# Autodesk Inventor assembly: Montagem1
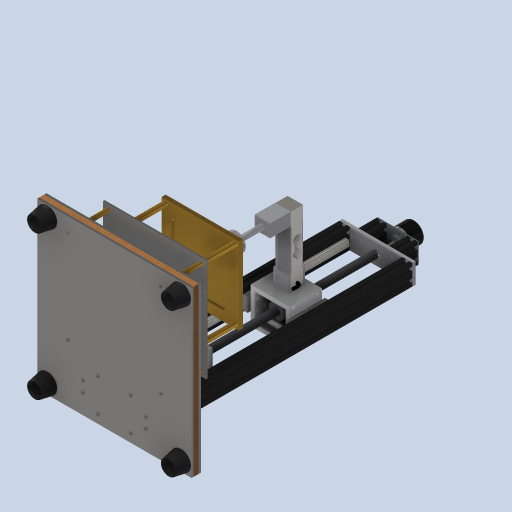
[picture p0: Inventor's stored thumbnail of the model, 512x512]
Saved by Autodesk Inventor 2023 (Build 270158000, 158)
## iProperties
Created: 2023-03-18
Part Number: Montagem1
Document SubType Name: Assembly
Designer: Mateus
Mass: 15449.6 g
Surface Area: 13309.4 cm^2
Volume: 3131.3 cm^3
Author: Mateus
## Documents named in this file (40)
- C:\Users\mateus\OneDrive - Fundação Salvador Arena\#TCC Texturômetro\1- Desenho mecânico\1-Modelagem\Texturômetro.iam
- C:\Users\mateus\OneDrive - Fundação Salvador Arena\#TCC Texturômetro\1- Desenho mecânico\1-Modelagem\Base.ipt
- C:\Users\mateus\OneDrive - Fundação Salvador Arena\#TCC Texturômetro\1- Desenho mecânico\1-Modelagem\Eixo roscado.ipt
- C:\Users\mateus\OneDrive - Fundação Salvador Arena\#TCC Texturômetro\1- Desenho mecânico\1-Modelagem\Motor.ipt
- C:\Users\mateus\OneDrive - Fundação Salvador Arena\#TCC Texturômetro\1- Desenho mecânico\1-Modelagem\Suporte do motor.ipt
- C:\Users\mateus\OneDrive - Fundação Salvador Arena\#TCC Texturômetro\1- Desenho mecânico\1-Modelagem\Sustentação motor.ipt
- C:\Users\mateus\OneDrive - Fundação Salvador Arena\#TCC Texturômetro\1- Desenho mecânico\1-Modelagem\Espaçador do motor.ipt
- C:\Users\mateus\OneDrive - Fundação Salvador Arena\#TCC Texturômetro\1- Desenho mecânico\1-Modelagem\Suporte inferior do eixo.ipt
- C:\Users\mateus\OneDrive - Fundação Salvador Arena\#TCC Texturômetro\1- Desenho mecânico\1-Modelagem\Suporte superior do eixo.ipt
- C:\Users\mateus\OneDrive - Fundação Salvador Arena\#TCC Texturômetro\1- Desenho mecânico\1-Modelagem\Suporte da base de apoio.ipt
- C:\Users\mateus\OneDrive - Fundação Salvador Arena\#TCC Texturômetro\1- Desenho mecânico\1-Modelagem\Base de apoio.ipt
- C:\Users\mateus\OneDrive - Fundação Salvador Arena\#TCC Texturômetro\1- Desenho mecânico\1-Modelagem\Guia do eixo roscado.ipt
- C:\Users\mateus\OneDrive - Fundação Salvador Arena\#TCC Texturômetro\1- Desenho mecânico\1-Modelagem\Suporte guia.ipt
- C:\Users\mateus\OneDrive - Fundação Salvador Arena\#TCC Texturômetro\1- Desenho mecânico\1-Modelagem\Guia do trilho.ipt
- C:\Users\mateus\OneDrive - Fundação Salvador Arena\#TCC Texturômetro\1- Desenho mecânico\1-Modelagem\Frente da caixa de sustentação.ipt
- C:\Users\mateus\OneDrive - Fundação Salvador Arena\#TCC Texturômetro\1- Desenho mecânico\1-Modelagem\Traseira da caixa de sustentação.ipt
- C:\Users\mateus\OneDrive - Fundação Salvador Arena\#TCC Texturômetro\1- Desenho mecânico\1-Modelagem\Suporte da célula de carga.ipt
- C:\Users\mateus\OneDrive - Fundação Salvador Arena\#TCC Texturômetro\1- Desenho mecânico\1-Modelagem\Suporte da probe.ipt
- C:\Users\mateus\OneDrive - Fundação Salvador Arena\#TCC Texturômetro\1- Desenho mecânico\1-Modelagem\Trilho.ipt
- C:\Users\mateus\OneDrive - Fundação Salvador Arena\#TCC Texturômetro\1- Desenho mecânico\1-Modelagem\Suporte base da mesa.ipt
- C:\Users\mateus\OneDrive - Fundação Salvador Arena\#TCC Texturômetro\1- Desenho mecânico\1-Modelagem\Suporte da mesa.ipt
- C:\Users\mateus\OneDrive - Fundação Salvador Arena\#TCC Texturômetro\1- Desenho mecânico\1-Modelagem\Placa da mesa.ipt
- C:\Users\mateus\OneDrive - Fundação Salvador Arena\#TCC Texturômetro\1- Desenho mecânico\1-Modelagem\Suporte mesa.ipt
- C:\Users\mateus\OneDrive - Fundação Salvador Arena\#TCC Texturômetro\1- Desenho mecânico\1-Modelagem\Probe.ipt
- C:\Users\mateus\OneDrive - Fundação Salvador Arena\#TCC Texturômetro\1- Desenho mecânico\1-Modelagem\Base madeira.ipt
- C:\Users\mateus\OneDrive - Fundação Salvador Arena\#TCC Texturômetro\1- Desenho mecânico\1-Modelagem\Perfil aluminio.ipt
- C:\Users\mateus\OneDrive - Fundação Salvador Arena\#TCC Texturômetro\1- Desenho mecânico\1-Modelagem\Lateral da caixa de sustentação.ipt
- C:\Users\mateus\OneDrive - Fundação Salvador Arena\#TCC Texturômetro\1- Desenho mecânico\1-Modelagem\Pés.ipt
- C:\Users\mateus\OneDrive - Fundação Salvador Arena\#TCC Texturômetro\1- Desenho mecânico\1-Modelagem\Perfil aluminio 2.ipt
- C:\Users\mateus\OneDrive - Fundação Salvador Arena\#TCC Texturômetro\1- Desenho mecânico\1-Modelagem\Suporte Encoder.ipt
- C:\Users\mateus\OneDrive - Fundação Salvador Arena\#TCC Texturômetro\1- Desenho mecânico\1-Modelagem\Encoder.ipt
- C:\Users\mateus\OneDrive - Fundação Salvador Arena\#TCC Texturômetro\1- Desenho mecânico\1-Modelagem\GLX-150_1.ipt
- C:\Users\mateus\OneDrive - Fundação Salvador Arena\#TCC Texturômetro\1- Desenho mecânico\1-Modelagem\Texturômetro\AIP\FEA\eaa23tyn4.fins
- C:\Users\mateus\OneDrive - Fundação Salvador Arena\#TCC Texturômetro\1- Desenho mecânico\1-Modelagem\Texturômetro\AIP\FEA\eaa23tyo0.fsat
- C:\Users\mateus\OneDrive - Fundação Salvador Arena\#TCC Texturômetro\1- Desenho mecânico\1-Modelagem\Texturômetro\AIP\FEA\eaa23tyo0.ftes
- C:\Users\mateus\OneDrive - Fundação Salvador Arena\#TCC Texturômetro\1- Desenho mecânico\1-Modelagem\Texturômetro\AIP\FEA\eaa23tyo0.fwiz
- C:\Users\mateus\OneDrive - Fundação Salvador Arena\#TCC Texturômetro\1- Desenho mecânico\1-Modelagem\Texturômetro\AIP\FEA\eaa23tytc.fmsh
- C:\Users\mateus\OneDrive - Fundação Salvador Arena\#TCC Texturômetro\1- Desenho mecânico\1-Modelagem\Texturômetro\AIP\FEA\ehg7firvk.fres
- C:\Users\mateus\OneDrive - Fundação Salvador Arena\#TCC Texturômetro\1- Desenho mecânico\1-Modelagem\Texturômetro\AIP\FEA\ei38k6pxc.fmsh
- C:\Users\mateus\OneDrive - Fundação Salvador Arena\#TCC Texturômetro\1- Desenho mecânico\1-Modelagem\Texturômetro\AIP\FEA\ei38k6pxd.fres
## Components (55 placed, 31 different names)
1. Base:1 — Coincidente:13, Coincidente:17, Alinhado:12, Coincidente:27, Coincidente:28, Coincidente:29, Coincidente:30, Coincidente:48, Alinhado:28, Alinhado:29, Coincidente:269, Alinhado:84, Coincidente:273, Alinhado:86, Coincidente:275, Flush:104, Mate:298
2. Eixo roscado:1 — Coincidente:13, Coincidente:49, Coincidente:248, Mate:285, Mate:293, Mate:294, Mate:296
3. Motor:1 — Mate:291, Mate:292, Angle:1, Mate:293, Mate:296
4. Suporte do motor:1 — Coincidente:31, Coincidente:32, Coincidente:33, Coincidente:34, Coincidente:35, Coincidente:36, Coincidente:37, Coincidente:38, Coincidente:39, Alinhado:22, Mate:117, Mate:291, Mate:292, Angle:1, Angle:2
5. Sustentação motor:1 — Coincidente:29, Coincidente:34, Mate:117
6. Sustentação motor:2 — Coincidente:27, Coincidente:33
7. Sustentação motor:3 — Coincidente:30, Coincidente:32
8. Sustentação motor:4 — Coincidente:28, Coincidente:31
9. Espaçador do motor:1 — Coincidente:35, Alinhado:19, Alinhado:20, Coincidente:39, Coincidente:41
10. Espaçador do motor:2 — Coincidente:36, Alinhado:20, Alinhado:21
11. Espaçador do motor:3 — Coincidente:38, Alinhado:19
12. Espaçador do motor:4 — Coincidente:37, Alinhado:21
13. Suporte inferior do eixo:1 — Alinhado:22, Coincidente:41, Mate:294
14. Suporte superior do eixo:1 — Coincidente:248, Alinhado:91, Coincidente:278, Mate:307, Mate:308, Mate:309, Mate:310, Mate:311, Mate:312
15. Suporte da base de apoio:1 — Coincidente:45, Alinhado:25, Alinhado:26
16. Suporte da base de apoio:2 — Alinhado:25, Coincidente:47, Coincidente:48, Mate:119
17. Suporte da base de apoio:3 — Coincidente:44, Alinhado:27
18. Suporte da base de apoio:4 — Coincidente:43, Alinhado:26, Alinhado:27
19. Base de apoio:1 — Coincidente:43, Coincidente:44, Coincidente:45, Coincidente:47, Alinhado:28, Alinhado:29, Alinhado:61, Alinhado:62, Mate:119, Mate:121
20. Guia do eixo roscado:1 — Coincidente:49, Coincidente:50, Coincidente:51
21. Suporte guia:1 — Coincidente:50, Coincidente:51, Mate:284, Flush:100
22. Guia do trilho:1 — Mate:60, Coincidente:206, Alinhado:74
23. Guia do trilho:2 — Mate:60, Flush:30, Coincidente:205, Alinhado:74, Alinhado:75, Coincidente:208, Mate:279
24. Guia do trilho:3 — Mate:61, Alinhado:72, Alinhado:73
25. Guia do trilho:4 — Mate:61, Flush:30, Alinhado:72, Alinhado:73, Coincidente:204, Alinhado:75, Mate:280, Flush:99
26. Frente da caixa de sustentação:2 — Mate:115, Coincidente:126, Flush:96, Flush:97, Mate:283, Angle:3
27. Traseira da caixa de sustentação:2 — Flush:94, Flush:95, Mate:281, Mate:282, Mate:284, Flush:100
28. Suporte da célula de carga:1 — Mate:115, Coincidente:126, Angle:3, Mate:319, Flush:105, Mate:320
29. Suporte da probe:1 — Mate:295, Mate:297, Mate:321, Flush:106, Mate:322
30. Trilho:1 — Alinhado:58, Alinhado:59, Coincidente:205, Coincidente:206, Coincidente:208, Coincidente:269, Coincidente:276
31. Trilho:2 — Alinhado:58, Alinhado:59, Coincidente:204, Coincidente:277, Alinhado:90
32. Suporte base da mesa:1 — Coincidente:106, Coincidente:107, Coincidente:108, Coincidente:109, Coincidente:110, Alinhado:61, Alinhado:62, Coincidente:111, Coincidente:112, Coincidente:113
33. Suporte da mesa:1 — Coincidente:108, Flush:67, Flush:68, Mate:125
34. Suporte da mesa:2 — Coincidente:106, Coincidente:110, Flush:68, Mate:123, Mate:124
35. Suporte da mesa:3 — Coincidente:109, Flush:66, Flush:67
36. Suporte da mesa:4 — Coincidente:107, Flush:66, Mate:122
37. Placa da mesa:1 — Coincidente:111, Coincidente:112, Coincidente:113
38. Suporte mesa:1 — Flush:69, Flush:70, Mate:121, Mate:122, Mate:123, Mate:124
39. Suporte mesa:2 — Flush:69, Flush:70, Mate:125
40. Probe:1 — Mate:295, Mate:297
41. Base madeira:1 — Alinhado:84, Alinhado:85, Coincidente:272, Coincidente:273, Alinhado:86, Alinhado:87, Flush:98, Angle:2, Mate:303, Mate:305
42. Base:2 — Alinhado:85, Coincidente:272, Alinhado:87, Mate:286, Mate:288, Mate:289, Mate:299, Mate:300, Mate:301, Mate:302, Mate:304
43. Perfil aluminio:1 — Alinhado:88, Alinhado:89, Coincidente:276, Flush:98, Mate:285
44. Perfil aluminio:2 — Alinhado:88, Alinhado:89, Coincidente:275, Coincidente:277, Alinhado:90, Alinhado:91, Coincidente:278
45. Lateral da caixa de sustentação:1 — Mate:279, Flush:92, Flush:93, Flush:94, Flush:95, Mate:281, Flush:96, Flush:97, Mate:283
46. Lateral da caixa de sustentação:2 — Mate:280, Flush:92, Flush:93, Mate:282, Flush:99
47. Pés:1 — Mate:300, Mate:305
48. Pés:2 — Mate:288, Flush:101, Mate:301, Mate:303
49. Pés:3 — Mate:286, Mate:298, Mate:299, Mate:306
50. Pés:4 — Mate:289, Flush:101, Flush:104, Mate:290, Mate:302, Mate:304
51. Perfil aluminio 2:1 — Mate:307, Mate:310, Mate:311, Mate:313, Mate:314
52. Perfil aluminio 2:2 — Mate:308, Mate:309, Mate:312, Mate:315
53. Suporte Encoder:1 — Mate:313, Mate:314, Mate:315, Mate:316, Mate:317, Mate:318
54. Encoder:1 — Mate:316, Mate:317, Mate:318
55. GLX-150_1:1 — Mate:319, Flush:105, Mate:320, Mate:321, Flush:106, Mate:322
## Relationships (146: Mate 98, Flush 45, Angle 3)
- Coincidente:13 [Mate] (-150 mm): Base:1 ↔ Eixo roscado:1
- Coincidente:17 [Mate]: Base:1
- Alinhado:12 [Flush]: Base:1
- Coincidente:27 [Mate]: Base:1 ↔ Sustentação motor:2
- Coincidente:28 [Mate]: Base:1 ↔ Sustentação motor:4
- Coincidente:29 [Mate]: Base:1 ↔ Sustentação motor:1
- Coincidente:30 [Mate]: Base:1 ↔ Sustentação motor:3
- Coincidente:31 [Mate]: Suporte do motor:1 ↔ Sustentação motor:4
- Coincidente:32 [Mate]: Suporte do motor:1 ↔ Sustentação motor:3
- Coincidente:33 [Mate]: Suporte do motor:1 ↔ Sustentação motor:2
- Coincidente:34 [Mate]: Suporte do motor:1 ↔ Sustentação motor:1
- Coincidente:35 [Mate]: Suporte do motor:1 ↔ Espaçador do motor:1
- Coincidente:36 [Mate]: Suporte do motor:1 ↔ Espaçador do motor:2
- Coincidente:37 [Mate]: Suporte do motor:1 ↔ Espaçador do motor:4
- Coincidente:38 [Mate]: Suporte do motor:1 ↔ Espaçador do motor:3
- Alinhado:19 [Flush]: Espaçador do motor:1 ↔ Espaçador do motor:3
- Alinhado:20 [Flush]: Espaçador do motor:1 ↔ Espaçador do motor:2
- Alinhado:21 [Flush]: Espaçador do motor:2 ↔ Espaçador do motor:4
- Coincidente:39 [Mate]: Suporte do motor:1 ↔ Espaçador do motor:1
- Alinhado:22 [Flush]: Suporte do motor:1 ↔ Suporte inferior do eixo:1
- Coincidente:41 [Mate]: Espaçador do motor:1 ↔ Suporte inferior do eixo:1
- Coincidente:43 [Mate]: Suporte da base de apoio:4 ↔ Base de apoio:1
- Coincidente:44 [Mate]: Suporte da base de apoio:3 ↔ Base de apoio:1
- Coincidente:45 [Mate]: Suporte da base de apoio:1 ↔ Base de apoio:1
- Alinhado:25 [Flush]: Suporte da base de apoio:1 ↔ Suporte da base de apoio:2
- Alinhado:26 [Flush]: Suporte da base de apoio:1 ↔ Suporte da base de apoio:4
- Alinhado:27 [Flush]: Suporte da base de apoio:3 ↔ Suporte da base de apoio:4
- Coincidente:47 [Mate]: Suporte da base de apoio:2 ↔ Base de apoio:1
- Coincidente:48 [Mate]: Base:1 ↔ Suporte da base de apoio:2
- Alinhado:28 [Flush] (50 mm): Base:1 ↔ Base de apoio:1
- Alinhado:29 [Flush] (18.1 mm): Base:1 ↔ Base de apoio:1
- Coincidente:49 [Mate]: Eixo roscado:1 ↔ Guia do eixo roscado:1
- Coincidente:50 [Mate]: Guia do eixo roscado:1 ↔ Suporte guia:1
- Coincidente:51 [Mate]: Guia do eixo roscado:1 ↔ Suporte guia:1
- Mate:60 (3 mm): Guia do trilho:1 ↔ Guia do trilho:2
- Mate:61 (3 mm): Guia do trilho:3 ↔ Guia do trilho:4
- Flush:30: Guia do trilho:2 ↔ Guia do trilho:4
- Alinhado:58 [Flush]: Trilho:1 ↔ Trilho:2
- Alinhado:59 [Flush]: Trilho:1 ↔ Trilho:2
- Coincidente:106 [Mate]: Suporte base da mesa:1 ↔ Suporte da mesa:2
- Coincidente:107 [Mate]: Suporte base da mesa:1 ↔ Suporte da mesa:4
- Coincidente:108 [Mate]: Suporte base da mesa:1 ↔ Suporte da mesa:1
- Coincidente:109 [Mate]: Suporte base da mesa:1 ↔ Suporte da mesa:3
- Coincidente:110 [Mate]: Suporte base da mesa:1 ↔ Suporte da mesa:2
- Alinhado:61 [Flush] (25 mm): Base de apoio:1 ↔ Suporte base da mesa:1
- Alinhado:62 [Flush] (25 mm): Base de apoio:1 ↔ Suporte base da mesa:1
- Coincidente:111 [Mate]: Suporte base da mesa:1 ↔ Placa da mesa:1
- Coincidente:112 [Mate]: Suporte base da mesa:1 ↔ Placa da mesa:1
- Coincidente:113 [Mate]: Suporte base da mesa:1 ↔ Placa da mesa:1
- Mate:115: Frente da caixa de sustentação:2 ↔ Suporte da célula de carga:1
- Mate:117: Suporte do motor:1 ↔ Sustentação motor:1
- Mate:119: Suporte da base de apoio:2 ↔ Base de apoio:1
- Flush:66: Suporte da mesa:3 ↔ Suporte da mesa:4
- Flush:67: Suporte da mesa:1 ↔ Suporte da mesa:3
- Flush:68: Suporte da mesa:1 ↔ Suporte da mesa:2
- Flush:69: Suporte mesa:1 ↔ Suporte mesa:2
- Flush:70: Suporte mesa:1 ↔ Suporte mesa:2
- Mate:121: Base de apoio:1 ↔ Suporte mesa:1
- Mate:122: Suporte da mesa:4 ↔ Suporte mesa:1
- Mate:123: Suporte da mesa:2 ↔ Suporte mesa:1
- Mate:124: Suporte da mesa:2 ↔ Suporte mesa:1
- Mate:125: Suporte da mesa:1 ↔ Suporte mesa:2
- Coincidente:126 [Mate]: Frente da caixa de sustentação:2 ↔ Suporte da célula de carga:1
- Alinhado:72 [Flush]: Guia do trilho:3 ↔ Guia do trilho:4
- Alinhado:73 [Flush]: Guia do trilho:3 ↔ Guia do trilho:4
- Coincidente:204 [Mate]: Guia do trilho:4 ↔ Trilho:2
- Coincidente:205 [Mate]: Guia do trilho:2 ↔ Trilho:1
- Coincidente:206 [Mate]: Guia do trilho:1 ↔ Trilho:1
- Alinhado:74 [Flush]: Guia do trilho:1 ↔ Guia do trilho:2
- Alinhado:75 [Flush]: Guia do trilho:2 ↔ Guia do trilho:4
- Coincidente:208 [Mate]: Guia do trilho:2 ↔ Trilho:1
- Coincidente:248 [Mate]: Eixo roscado:1 ↔ Suporte superior do eixo:1
- Coincidente:269 [Mate] (12.5 mm): Base:1 ↔ Trilho:1
- Alinhado:84 [Flush]: Base:1 ↔ Base madeira:1
- Alinhado:85 [Flush]: Base madeira:1 ↔ Base:2
- Coincidente:272 [Mate]: Base madeira:1 ↔ Base:2
- Coincidente:273 [Mate]: Base:1 ↔ Base madeira:1
- Alinhado:86 [Flush]: Base:1 ↔ Base madeira:1
- Alinhado:87 [Flush]: Base madeira:1 ↔ Base:2
- Alinhado:88 [Flush]: Perfil aluminio:1 ↔ Perfil aluminio:2
- Alinhado:89 [Flush]: Perfil aluminio:1 ↔ Perfil aluminio:2
- Coincidente:275 [Mate]: Base:1 ↔ Perfil aluminio:2
- Coincidente:276 [Mate]: Trilho:1 ↔ Perfil aluminio:1
- Coincidente:277 [Mate]: Trilho:2 ↔ Perfil aluminio:2
- Alinhado:90 [Flush] (14 mm): Trilho:2 ↔ Perfil aluminio:2
- Alinhado:91 [Flush]: Suporte superior do eixo:1 ↔ Perfil aluminio:2
- Coincidente:278 [Mate]: Suporte superior do eixo:1 ↔ Perfil aluminio:2
- Mate:279: Guia do trilho:2 ↔ Lateral da caixa de sustentação:1
- Mate:280: Guia do trilho:4 ↔ Lateral da caixa de sustentação:2
- Flush:92: Lateral da caixa de sustentação:1 ↔ Lateral da caixa de sustentação:2
- Flush:93: Lateral da caixa de sustentação:1 ↔ Lateral da caixa de sustentação:2
- Flush:94: Traseira da caixa de sustentação:2 ↔ Lateral da caixa de sustentação:1
- Flush:95: Traseira da caixa de sustentação:2 ↔ Lateral da caixa de sustentação:1
- Mate:281: Traseira da caixa de sustentação:2 ↔ Lateral da caixa de sustentação:1
- Mate:282: Traseira da caixa de sustentação:2 ↔ Lateral da caixa de sustentação:2
- Flush:96: Frente da caixa de sustentação:2 ↔ Lateral da caixa de sustentação:1
- Flush:97: Frente da caixa de sustentação:2 ↔ Lateral da caixa de sustentação:1
- Mate:283: Frente da caixa de sustentação:2 ↔ Lateral da caixa de sustentação:1
- Mate:284: Suporte guia:1 ↔ Traseira da caixa de sustentação:2
- Flush:98 (28.4 mm): Base madeira:1 ↔ Perfil aluminio:1
- Flush:99 (5.25 mm): Guia do trilho:4 ↔ Lateral da caixa de sustentação:2
- Mate:285 (51 mm): Eixo roscado:1 ↔ Perfil aluminio:1
- Flush:100 (9.25 mm): Suporte guia:1 ↔ Traseira da caixa de sustentação:2
- Mate:286: Base:2 ↔ Pés:3
- Mate:288: Base:2 ↔ Pés:2
- Mate:289: Base:2 ↔ Pés:4
- Flush:101: Pés:2 ↔ Pés:4
- Flush:104: Base:1 ↔ Pés:4
- Mate:290: Pés:4
- Mate:291: Motor:1 ↔ Suporte do motor:1
- Mate:292: Motor:1 ↔ Suporte do motor:1
- Angle:1 (0 deg): Motor:1 ↔ Suporte do motor:1
- Mate:293: Eixo roscado:1 ↔ Motor:1
- Mate:294: Eixo roscado:1 ↔ Suporte inferior do eixo:1
- Angle:2 (0 deg): Suporte do motor:1 ↔ Base madeira:1
- Mate:295: Suporte da probe:1 ↔ Probe:1
- Mate:296 (8 mm): Eixo roscado:1 ↔ Motor:1
- Angle:3 (0 deg): Frente da caixa de sustentação:2 ↔ Suporte da célula de carga:1
- Mate:297: Suporte da probe:1 ↔ Probe:1
- Mate:298: Base:1 ↔ Pés:3
- Mate:299: Base:2 ↔ Pés:3
- Mate:300: Base:2 ↔ Pés:1
- Mate:301: Base:2 ↔ Pés:2
- Mate:302: Base:2 ↔ Pés:4
- Mate:303: Base madeira:1 ↔ Pés:2
- Mate:304: Base:2 ↔ Pés:4
- Mate:305: Base madeira:1 ↔ Pés:1
- Mate:306: Pés:3
- Mate:307: Suporte superior do eixo:1 ↔ Perfil aluminio 2:1
- Mate:308: Suporte superior do eixo:1 ↔ Perfil aluminio 2:2
- Mate:309: Suporte superior do eixo:1 ↔ Perfil aluminio 2:2
- Mate:310: Suporte superior do eixo:1 ↔ Perfil aluminio 2:1
- Mate:311: Suporte superior do eixo:1 ↔ Perfil aluminio 2:1
- Mate:312: Suporte superior do eixo:1 ↔ Perfil aluminio 2:2
- Mate:313: Perfil aluminio 2:1 ↔ Suporte Encoder:1
- Mate:314: Perfil aluminio 2:1 ↔ Suporte Encoder:1
- Mate:315: Perfil aluminio 2:2 ↔ Suporte Encoder:1
- Mate:316: Suporte Encoder:1 ↔ Encoder:1
- Mate:317: Suporte Encoder:1 ↔ Encoder:1
- Mate:318: Suporte Encoder:1 ↔ Encoder:1
- Mate:319: Suporte da célula de carga:1 ↔ GLX-150_1:1
- Flush:105: Suporte da célula de carga:1 ↔ GLX-150_1:1
- Mate:320: Suporte da célula de carga:1 ↔ GLX-150_1:1
- Mate:321: Suporte da probe:1 ↔ GLX-150_1:1
- Flush:106: Suporte da probe:1 ↔ GLX-150_1:1
- Mate:322: Suporte da probe:1 ↔ GLX-150_1:1
## Named parameters: sa_0 = 10000, sa_1 = 10000, sa_2 = 10000
note: some values were not read from the file. Shown as the stored number, unit unknown: "sa_0", "sa_1", "sa_2".
